# Autodesk Inventor assembly: 6Plaction-asm V2
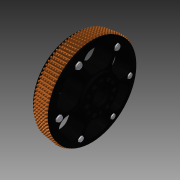
[picture p0: Inventor's stored thumbnail of the model, 180x180]
Saved by Autodesk Inventor 2014 SP1 (Build 180222100, 222)
## iProperties
Created: 2013-01-17
Part Number: 6Plaction-asm V2
Document SubType Name: Assembly
Designer: Moses
Mass: 367.41 g
Surface Area: 1346.56 cm^2
Volume: 310.737 cm^3
Density: 1.18238 g/cm^3
Author: Moses
## Documents named in this file (5)
- C:\Users\Moses\Documents\Inventor\Sally Rebuild\Rebuild Sally\6Plaction-asm V2.iam
- C:\Users\Moses\Documents\Inventor\Sally Rebuild\Rebuild Sally\6MW_d01.ipt
- C:\Users\Moses\Documents\Inventor\Sally Rebuild\Rebuild Sally\10-32x1000shcs.ipt
- C:\Users\Moses\Documents\Inventor\Sally Rebuild\Rebuild Sally\10-32_locknut.ipt
- C:\Users\Moses\Documents\Inventor\Sally Rebuild\Rebuild Sally\Plaction Tread 6-Inch Wheel V2.ipt
## Components (15 placed, 4 different names)
1. 6MW_d01:1 — Mate:2, Mate:3, Mate:4, Mate:5
2. 6MW_d01:2 — Mate:1, Mate:3, Mate:4, Mate:5
3. 10-32x1000shcs:1
4. 10-32x1000shcs:2
5. 10-32x1000shcs:3
6. 10-32x1000shcs:4
7. 10-32x1000shcs:5
8. 10-32x1000shcs:6
9. 10-32_locknut:1
10. 10-32_locknut:2
11. 10-32_locknut:3
12. 10-32_locknut:4
13. 10-32_locknut:5
14. 10-32_locknut:6
15. Plaction Tread 6-Inch Wheel V2:1 — Mate:1, Mate:2
## Relationships (5: Mate 5)
- Mate:1: 6MW_d01:2 ↔ Plaction Tread 6-Inch Wheel V2:1
- Mate:2: 6MW_d01:1 ↔ Plaction Tread 6-Inch Wheel V2:1
- Mate:3: 6MW_d01:1 ↔ 6MW_d01:2
- Mate:4: 6MW_d01:1 ↔ 6MW_d01:2
- Mate:5: 6MW_d01:1 ↔ 6MW_d01:2
